# Autodesk Inventor assembly: 知能ロボコン合体２
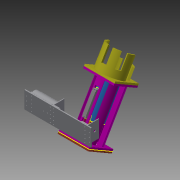
[picture p0: Inventor's stored thumbnail of the model, 180x180]
Saved by Autodesk Inventor 2013 (Build 170138000, 138)
## iProperties
Created: 2014-05-21
Part Number: 知能ロボコン合体２
Document SubType Name: Assembly
Designer: horumo136
Author: horumo136
## Documents named in this file (6)
- C:\Users\horumo136\Documents\知能ロボコン合体２.iam
- C:\Users\horumo136\Documents\セクターギア支え.ipt
- C:\Users\horumo136\Documents\知能ロボコンＬ字.ipt
- C:\Users\horumo136\Documents\タミヤ遊星ギアセット.ipt
- C:\Users\horumo136\Documents\知能ロボコン敷板.ipt
- C:\Users\horumo136\Documents\知能ロボコン合体１.iam
## Components (6 placed, 5 different names)
1. セクターギア支え:1 — メイト:5, メイト:6, メイト:7, メイト:8, メイト:9, メイト:10, メイト:11, メイト:12, メイト:13, メイト:17, メイト:18, メイト:19
2. 知能ロボコンＬ字:1 — メイト:5, メイト:6, メイト:7
3. 知能ロボコンＬ字:2 — メイト:8, メイト:9, メイト:10
4. タミヤ遊星ギアセット:1 — メイト:14, メイト:15, メイト:16
5. 知能ロボコン敷板:1 — メイト:11, メイト:12, メイト:13, メイト:14, メイト:15, メイト:16
6. 知能ロボコン合体１:1 [sub-assembly] — メイト:17, メイト:18, メイト:19
## Relationships (15: Mate 15)
- メイト:5 [Mate]: セクターギア支え:1 ↔ 知能ロボコンＬ字:1
- メイト:6 [Mate]: セクターギア支え:1 ↔ 知能ロボコンＬ字:1
- メイト:7 [Mate]: セクターギア支え:1 ↔ 知能ロボコンＬ字:1
- メイト:8 [Mate]: セクターギア支え:1 ↔ 知能ロボコンＬ字:2
- メイト:9 [Mate]: セクターギア支え:1 ↔ 知能ロボコンＬ字:2
- メイト:10 [Mate]: セクターギア支え:1 ↔ 知能ロボコンＬ字:2
- メイト:11 [Mate]: セクターギア支え:1 ↔ 知能ロボコン敷板:1
- メイト:12 [Mate]: セクターギア支え:1 ↔ 知能ロボコン敷板:1
- メイト:13 [Mate]: セクターギア支え:1 ↔ 知能ロボコン敷板:1
- メイト:14 [Mate]: タミヤ遊星ギアセット:1 ↔ 知能ロボコン敷板:1
- メイト:15 [Mate]: タミヤ遊星ギアセット:1 ↔ 知能ロボコン敷板:1
- メイト:16 [Mate]: タミヤ遊星ギアセット:1 ↔ 知能ロボコン敷板:1
- メイト:17 [Mate]: セクターギア支え:1 ↔ 知能ロボコン合体１:1
- メイト:18 [Mate]: セクターギア支え:1 ↔ 知能ロボコン合体１:1
- メイト:19 [Mate]: セクターギア支え:1 ↔ 知能ロボコン合体１:1
